# Autodesk Inventor assembly: pld_nipple-70mm
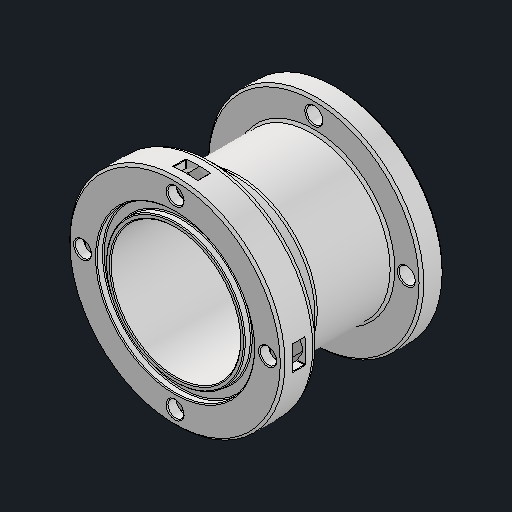
[picture p0: Inventor's stored thumbnail of the model, 512x512]
Saved by Autodesk Inventor 2026 (Build 300175050, 175E)
## iProperties
Created: 2025-12-03
Part Number: pld_nipple-70mm
Document SubType Name: Assembly
Designer: queezz
Author: queezz
## Documents named in this file (3)
- C:\Users\queezz\Dropbox\Drawings\PIHTI\PLD\pld_nipple-70mm.iam
- C:\Users\queezz\Dropbox\Drawings\PIHTI\PLD\pld_nipple_60mm.ipt
- C:\Users\queezz\Dropbox\Drawings\PIHTI\ContentCenter\Fastners\M6-nut-WA5.ipt
## Components (5 placed, 2 different names)
1. pld_nipple_60mm:1 — Rigid:1, Rigid:2, Rigid:3, Rigid:4
2. JIS B 1181 -finished Class 1 - Metric Class 1 -finishedM6:1 — Rigid:3
3. JIS B 1181 -finished Class 1 - Metric Class 1 -finishedM6:2 — Rigid:4
4. JIS B 1181 -finished Class 1 - Metric Class 1 -finishedM6:3 — Rigid:2
5. JIS B 1181 -finished Class 1 - Metric Class 1 -finishedM6:4 — Rigid:1
## Relationships (4: WeldJoint 4)
- Rigid:1 [WeldJoint]: pld_nipple_60mm:1 ↔ JIS B 1181 -finished Class 1 - Metric Class 1 -finishedM6:4
- Rigid:2 [WeldJoint]: pld_nipple_60mm:1 ↔ JIS B 1181 -finished Class 1 - Metric Class 1 -finishedM6:3
- Rigid:3 [WeldJoint]: pld_nipple_60mm:1 ↔ JIS B 1181 -finished Class 1 - Metric Class 1 -finishedM6:1
- Rigid:4 [WeldJoint]: pld_nipple_60mm:1 ↔ JIS B 1181 -finished Class 1 - Metric Class 1 -finishedM6:2
